# Autodesk Inventor assembly: 552198 EMGA-120-P-G3-SAS-140
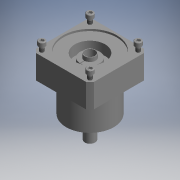
[picture p0: Inventor's stored thumbnail of the model, 180x180]
Saved by Autodesk Inventor 2017.3 (Build 213256000, 256)
## iProperties
Category: PARTsolutions
Company: FESTO
Part Number: 552198 EMGA-120-P-G3-SAS-140
Catalog Web Link: www.cadenas.de
Description: EMGA-gear unit
Vendor: FESTO
Document SubType Name: Assembly
Designer: partserver
Manufacturer: FESTO
Mass: 6000 g
Surface Area: 1288.55 cm^2
Volume: 1787.97 cm^3
Density: 3.35576 g/cm^3
Title: 552198 EMGA-120-P-G3-SAS-140
Author: Cadenas PARTsolutions
Comments: gear unit
PSOL_IDENT_0: {ATYP=ASSISTANT},{DATA=script=$CADENAS_DATA/23d-libs/festo/webfesto.vbb&M_FAMILY=EMGA&M_GROUP=01&M_P
PSOL_IDENT_1: ARTNO=552198&IDCODE1=EMGA-120-P-G3-SAS-140&IDCODE2=&customer_number_cns=&MATES=1&LOD=HI&LOCKERP=0&SI
PSOL_IDENT_2: NGLEPART=1}
NB: 552198 EMGA-120-P-G3-SAS-140
NN: EMGA
NT: gear unit
NBSYN: $TNR. $TYP.
LINA: 552198 EMGA-120-P-G3-SAS-140
CATALOG: Festo
TNR: 552198
TYP: EMGA-120-P-G3-SAS-140
CNSMASSEXACT: 6
SUPPLIER: FESTO
ARTICLENO: 552198 EMGA-120-P-G3-SAS-140
BOMINFO: 552198 EMGA-120-P-G3-SAS-140
CREATOR: CADENAS GmbH
## Documents named in this file (3)
- e:\temp\worker_27\temp\exporttempdir_9356_16_uyLlD\format_0\552198 EMGA-120-P-G3-SAS-140.iam
- e:\temp\worker_27\temp\exporttempdir_9356_16_uyLlD\format_0\552198 EMGA-120-P-G3-SAS-140---(P).ipt
- e:\temp\worker_27\temp\exporttempdir_9356_16_uyLlD\format_0\DIN-912 - M10x35(F).ipt
## Components (5 placed, 2 different names)
1. 552198 EMGA-120-P-G3-SAS-140---(P):1 — S_1_XY@1 <-> ANBAU_XY@2, S_1_Z@1 <-> ANBAU_Z@2, S_1_YZ@1 <-> ANBAU_YZ@2, S_2_XY@1 <-> ANBAU_XY@3, S_2_Z@1 <-> ANBAU_Z@3, S_2_YZ@1 <-> ANBAU_YZ@3, S_3_XY@1 <-> ANBAU_XY@4, S_3_Z@1 <-> ANBAU_Z@4, S_3_YZ@1 <-> ANBAU_YZ@4, S_4_XY@1 <-> ANBAU_XY@5, S_4_Z@1 <-> ANBAU_Z@5, S_4_YZ@1 <-> ANBAU_YZ@5
2. DIN-912 - M10x35(F):1 — S_1_XY@1 <-> ANBAU_XY@2, S_1_Z@1 <-> ANBAU_Z@2, S_1_YZ@1 <-> ANBAU_YZ@2
3. DIN-912 - M10x35(F):2 — S_2_XY@1 <-> ANBAU_XY@3, S_2_Z@1 <-> ANBAU_Z@3, S_2_YZ@1 <-> ANBAU_YZ@3
4. DIN-912 - M10x35(F):3 — S_3_XY@1 <-> ANBAU_XY@4, S_3_Z@1 <-> ANBAU_Z@4, S_3_YZ@1 <-> ANBAU_YZ@4
5. DIN-912 - M10x35(F):4 — S_4_XY@1 <-> ANBAU_XY@5, S_4_Z@1 <-> ANBAU_Z@5, S_4_YZ@1 <-> ANBAU_YZ@5
## Relationships (12: Flush 4, Mate 4, Angle 4)
- S_1_XY@1 <-> ANBAU_XY@2 [Flush]: 552198 EMGA-120-P-G3-SAS-140---(P):1 ↔ DIN-912 - M10x35(F):1
- S_1_Z@1 <-> ANBAU_Z@2 [Mate]: 552198 EMGA-120-P-G3-SAS-140---(P):1 ↔ DIN-912 - M10x35(F):1
- S_1_YZ@1 <-> ANBAU_YZ@2 [Angle] (0 deg): 552198 EMGA-120-P-G3-SAS-140---(P):1 ↔ DIN-912 - M10x35(F):1
- S_2_XY@1 <-> ANBAU_XY@3 [Flush]: 552198 EMGA-120-P-G3-SAS-140---(P):1 ↔ DIN-912 - M10x35(F):2
- S_2_Z@1 <-> ANBAU_Z@3 [Mate]: 552198 EMGA-120-P-G3-SAS-140---(P):1 ↔ DIN-912 - M10x35(F):2
- S_2_YZ@1 <-> ANBAU_YZ@3 [Angle] (0 deg): 552198 EMGA-120-P-G3-SAS-140---(P):1 ↔ DIN-912 - M10x35(F):2
- S_3_XY@1 <-> ANBAU_XY@4 [Flush]: 552198 EMGA-120-P-G3-SAS-140---(P):1 ↔ DIN-912 - M10x35(F):3
- S_3_Z@1 <-> ANBAU_Z@4 [Mate]: 552198 EMGA-120-P-G3-SAS-140---(P):1 ↔ DIN-912 - M10x35(F):3
- S_3_YZ@1 <-> ANBAU_YZ@4 [Angle] (0 deg): 552198 EMGA-120-P-G3-SAS-140---(P):1 ↔ DIN-912 - M10x35(F):3
- S_4_XY@1 <-> ANBAU_XY@5 [Flush]: 552198 EMGA-120-P-G3-SAS-140---(P):1 ↔ DIN-912 - M10x35(F):4
- S_4_Z@1 <-> ANBAU_Z@5 [Mate]: 552198 EMGA-120-P-G3-SAS-140---(P):1 ↔ DIN-912 - M10x35(F):4
- S_4_YZ@1 <-> ANBAU_YZ@5 [Angle] (0 deg): 552198 EMGA-120-P-G3-SAS-140---(P):1 ↔ DIN-912 - M10x35(F):4
